# Autodesk Inventor assembly: CABEZAL
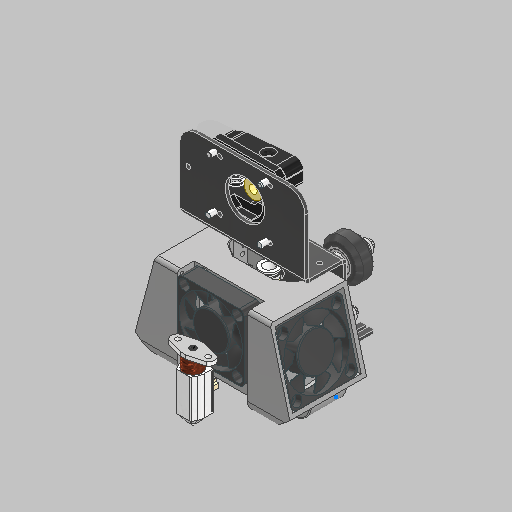
[picture p0: Inventor's stored thumbnail of the model, 512x512]
Saved by Autodesk Inventor 2025.4 (Build 294407000, 407)
## iProperties
Created: 2025-10-28
Part Number: CABEZAL
Document SubType Name: Assembly
Designer: Inema
Author: Inema
## Documents named in this file (6)
- C:\Users\Inema\OneDrive\GitHub\Ender-3\Ender-3 Mechanical\Modificada\CABEZAL.iam
- C:\Users\Inema\OneDrive\GitHub\Ender-3\Ender-3 Mechanical\Modificada\ASM Extruder.iam
- C:\Users\Inema\OneDrive\GitHub\Ender-3\Ender-3 Mechanical\Modificada\ASM Printing Head.iam
- C:\Users\Inema\OneDrive\GitHub\Ender-3\Ender-3 Mechanical\Modificada\mS_Ender_Dual_4010_1.1\mS_Ender_Dual_4010_1.1\mS_Ender_Dual_4010_1.1.ipt
- C:\Users\Inema\OneDrive\GitHub\Ender-3\Ender-3 Mechanical\Modificada\Nozzle fan.ipt
- C:\Users\Inema\OneDrive\GitHub\Ender-3\Ender-3 Mechanical\Modificada\3d-touch-v30.ipt
## Components (7 placed, 6 different names)
1. ASM Extruder_162 [sub-assembly]
2. ASM Printing Head_167 [sub-assembly] — Insertar:1, Coincidencia:2
3. mS_Ender_Dual_4010_1.1:1 — Insertar:1, Coincidencia:2
4. Nozzle fan_172
5. Nozzle fan:2
6. Nozzle fan:3
7. 3d-touch-v30:1
## Relationships (5: Mate 2, Angle 1, Flush 1, Insert 1)
- [Mate]: ASM Extruder_162 ↔ ASM Printing Head_167
- [Angle] (180 deg): ASM Extruder_162 ↔ ASM Printing Head_167
- [Flush] (-1.45 mm): ASM Extruder_162 ↔ ASM Printing Head_167
- Insertar:1: ASM Printing Head_167 ↔ mS_Ender_Dual_4010_1.1:1
- Coincidencia:2 [Mate]: ASM Printing Head_167 ↔ mS_Ender_Dual_4010_1.1:1
